# Autodesk Inventor assembly: MG-Jetson
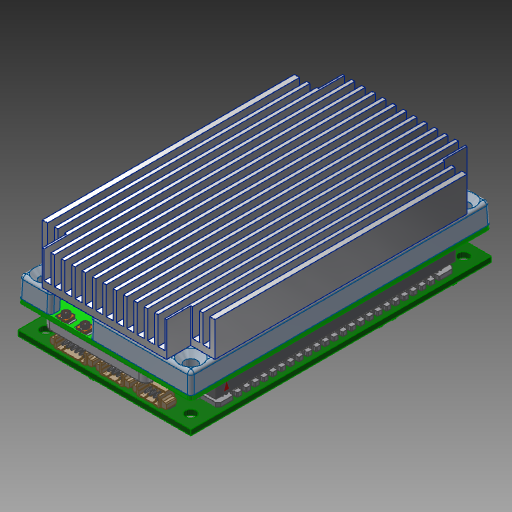
[picture p0: Inventor's stored thumbnail of the model, 512x512]
Saved by Autodesk Inventor 2019.4 (Build 234330000, 330)
## iProperties
Part Number: MG-Jetson
Material: Generisch
Document SubType Name: Assembly
Designer: rYan
Mass: 89.5888 g
Surface Area: 941.236 cm^2
Volume: 55.31 cm^3
Density: 1.61976 g/cm^3
Author: rYan
## Documents named in this file (4)
- D:\TIGERsGIT\Hardware\mechanik\2020\Inventor\Elektronik\MG-Jetson.iam
- D:\TIGERsGIT\Hardware\mechanik\2020\Inventor\Kaufteile\Auvidea J100 38188-2.ipt
- D:\TIGERsGIT\Hardware\mechanik\2020\Inventor\Kaufteile\Jetson TX2 Module.ipt
- D:\TIGERsGIT\Hardware\mechanik\2020\Inventor\Kaufteile\Jetson Kühlkörper Original.ipt
## Components (3 placed, 3 different names)
1. Auvidea J100 38188-2:1
2. Jetson TX2 Module:1 — Passend:2, Fluchtend:3, Fluchtend:4, Passend:3, Fluchtend:5, Fluchtend:6
3. Jetson Kühlkörper:1 — Passend:3, Fluchtend:5, Fluchtend:6
## Relationships (9: Flush 6, Mate 3)
- [Flush]: Auvidea J100 38188-2:1 ↔ Jetson TX2 Module:1
- [Flush]: Auvidea J100 38188-2:1 ↔ Jetson TX2 Module:1
- [Mate] (7 mm): Auvidea J100 38188-2:1 ↔ Jetson TX2 Module:1
- Passend:2 [Mate]: Jetson TX2 Module:1
- Fluchtend:3 [Flush]: Jetson TX2 Module:1
- Fluchtend:4 [Flush]: Jetson TX2 Module:1
- Passend:3 [Mate]: Jetson TX2 Module:1 ↔ Jetson Kühlkörper:1
- Fluchtend:5 [Flush]: Jetson TX2 Module:1 ↔ Jetson Kühlkörper:1
- Fluchtend:6 [Flush]: Jetson TX2 Module:1 ↔ Jetson Kühlkörper:1
